# Autodesk Inventor assembly: prig to kauri conversion
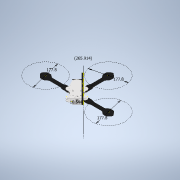
[picture p0: Inventor's stored thumbnail of the model, 180x180]
Saved by Autodesk Inventor 2020 (Build 240168000, 168)
## iProperties
Created: 2022-05-24
Part Number: prig to kauri conversion
Document SubType Name: Assembly
Designer: Steven
Author: Steven
## Documents named in this file (8)
- Y:\FPV drone stuff\0 Street League\Frames\experimental-quad-frames\prig to kauri conversion.iam
- Y:\FPV drone stuff\0 Street League\Frames\experimental-quad-frames\Kauri arm disc aero.ipt
- Y:\FPV drone stuff\0 Street League\Frames\experimental-quad-frames\399 prig z plate.ipt
- Y:\FPV drone stuff\0 Street League\Frames\PB-Kauri-X\Kauri side plate.ipt
- Y:\FPV drone stuff\0 Street League\Frames\PB-Kauri-X\3D prints\35 mm canopy\KauriRearLink 35mm no brass insert.ipt
- Y:\FPV drone stuff\0 Street League\Frames\experimental-quad-frames\prig to kauri conversion plate.ipt
- Y:\FPV drone stuff\0 Street League\Frames\experimental-quad-frames\prig to kauri conversion front link.ipt
- Y:\FPV drone stuff\0 Street League\Frames\experimental-quad-frames\hobbywingStack30_v1.ipt
## Components (13 placed, 7 different names)
1. Kauri arm disc aero:1 — Flush:1, Flush:2, Flush:3, Mate:1, Mate:2, Mate:3
2. Kauri arm disc aero:2 — Flush:1, Mate:4, Mate:5, Mate:10
3. Kauri arm disc aero:3 — Flush:2, Mate:6, Mate:7, Mate:12
4. Kauri arm disc aero:4 — Flush:3, Mate:8, Mate:9, Mate:11
5. 399 prig z plate:1 — Mate:1, Mate:2, Mate:3, Mate:4, Mate:5, Mate:6, Mate:7, Mate:8, Mate:9, Mate:23, Mate:24, Mate:25
6. 399 prig z plate:2 — Mate:10, Mate:11, Mate:12, Flush:4, Mate:16, Mate:17, Mate:18, Mate:20, Mate:21, Mate:22, Mate:30, Mate:31, Mate:32
7. Kauri side plate:1 — Mate:13, Mate:14, Mate:15, Flush:4
8. Kauri side plate:2 — Mate:13, Mate:14, Mate:15, Mate:19, Mate:29
9. KauriRearLink 35mm no brass insert:1 — Mate:16, Mate:17, Mate:18, Mate:19
10. prig to kauri conversion plate:1 — Mate:20, Mate:21, Mate:22, Mate:28
11. prig to kauri conversion plate:2 — Mate:23, Mate:24, Mate:25, Mate:26, Mate:27
12. prig to kauri conversion front link:1 — Mate:26, Mate:27, Mate:28, Mate:29
13. hobbywingStack30_v1:1 — Mate:30, Mate:31, Mate:32
## Relationships (36: Mate 32, Flush 4)
- Flush:1: Kauri arm disc aero:1 ↔ Kauri arm disc aero:2
- Flush:2: Kauri arm disc aero:1 ↔ Kauri arm disc aero:3
- Flush:3: Kauri arm disc aero:1 ↔ Kauri arm disc aero:4
- Mate:1: Kauri arm disc aero:1 ↔ 399 prig z plate:1
- Mate:2: Kauri arm disc aero:1 ↔ 399 prig z plate:1
- Mate:3: Kauri arm disc aero:1 ↔ 399 prig z plate:1
- Mate:4: Kauri arm disc aero:2 ↔ 399 prig z plate:1
- Mate:5: Kauri arm disc aero:2 ↔ 399 prig z plate:1
- Mate:6: Kauri arm disc aero:3 ↔ 399 prig z plate:1
- Mate:7: Kauri arm disc aero:3 ↔ 399 prig z plate:1
- Mate:8: Kauri arm disc aero:4 ↔ 399 prig z plate:1
- Mate:9: Kauri arm disc aero:4 ↔ 399 prig z plate:1
- Mate:10: Kauri arm disc aero:2 ↔ 399 prig z plate:2
- Mate:11: Kauri arm disc aero:4 ↔ 399 prig z plate:2
- Mate:12: Kauri arm disc aero:3 ↔ 399 prig z plate:2
- Mate:13: Kauri side plate:1 ↔ Kauri side plate:2
- Mate:14: Kauri side plate:1 ↔ Kauri side plate:2
- Mate:15 (35 mm): Kauri side plate:1 ↔ Kauri side plate:2
- Flush:4 (7.5 mm): 399 prig z plate:2 ↔ Kauri side plate:1
- Mate:16: 399 prig z plate:2 ↔ KauriRearLink 35mm no brass insert:1
- Mate:17: 399 prig z plate:2 ↔ KauriRearLink 35mm no brass insert:1
- Mate:18: 399 prig z plate:2 ↔ KauriRearLink 35mm no brass insert:1
- Mate:19: Kauri side plate:2 ↔ KauriRearLink 35mm no brass insert:1
- Mate:20: 399 prig z plate:2 ↔ prig to kauri conversion plate:1
- Mate:21: 399 prig z plate:2 ↔ prig to kauri conversion plate:1
- Mate:22: 399 prig z plate:2 ↔ prig to kauri conversion plate:1
- Mate:23: 399 prig z plate:1 ↔ prig to kauri conversion plate:2
- Mate:24: 399 prig z plate:1 ↔ prig to kauri conversion plate:2
- Mate:25: 399 prig z plate:1 ↔ prig to kauri conversion plate:2
- Mate:26: prig to kauri conversion plate:2 ↔ prig to kauri conversion front link:1
- Mate:27: prig to kauri conversion plate:2 ↔ prig to kauri conversion front link:1
- Mate:28: prig to kauri conversion plate:1 ↔ prig to kauri conversion front link:1
- Mate:29: Kauri side plate:2 ↔ prig to kauri conversion front link:1
- Mate:30: 399 prig z plate:2 ↔ hobbywingStack30_v1:1
- Mate:31: 399 prig z plate:2 ↔ hobbywingStack30_v1:1
- Mate:32: 399 prig z plate:2 ↔ hobbywingStack30_v1:1
